# Autodesk Inventor assembly: embasev2
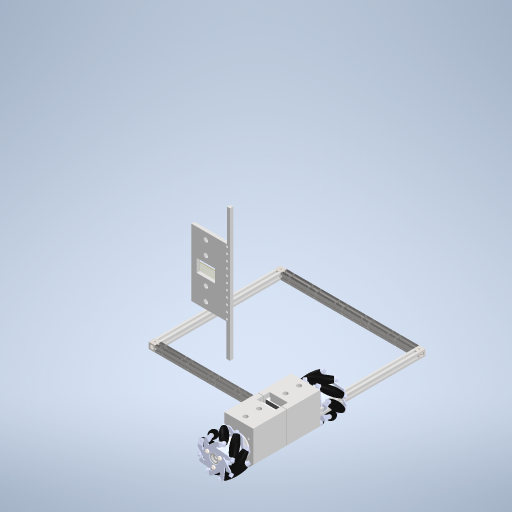
[picture p0: Inventor's stored thumbnail of the model, 512x512]
Saved by Autodesk Inventor 2024.2 (Build 282272000, 272)
## iProperties
Created: 2023-12-11
Part Number: embasev2
Document SubType Name: Assembly
Designer: adrie
Author: adrie
## Documents named in this file (24)
- C:\Users\eleves\Desktop\meca_robotbebou\embasev2\embasev2.iam
- C:\Users\eleves\Desktop\meca_robotbebou\embasev2\support_moteur_v3.ipt
- C:\Users\eleves\Desktop\meca_robotbebou\SF2423-10B41_MIR1.ipt
- C:\Users\eleves\Desktop\meca_robotbebou\60mm Double Aluminum Mecanum Wheel_MIR1.ipt
- C:\Users\eleves\Desktop\meca_robotbebou\moyeu_MIR1.ipt
- C:\Users\eleves\Desktop\meca_robotbebou\moyeu_end_MIR1.ipt
- C:\Users\eleves\Desktop\meca_robotbebou\embasev2\support_moteur_v3_MIR.ipt
- C:\Users\eleves\Desktop\meca_robotbebou\SF2423-10B41_MIR1_MIR.ipt
- C:\Users\eleves\Desktop\meca_robotbebou\60mm Double Aluminum Mecanum Wheel_MIR1_MIR.ipt
- C:\Users\eleves\Desktop\meca_robotbebou\moyeu_MIR1_MIR.ipt
- C:\Users\eleves\Desktop\meca_robotbebou\moyeu_end_MIR1_MIR.ipt
- C:\Users\eleves\Desktop\meca_robotbebou\SF2423-10B41_MIR1_MIR3.ipt
- C:\Users\eleves\Desktop\meca_robotbebou\60mm Double Aluminum Mecanum Wheel_MIR1_MIR3.ipt
- C:\Users\eleves\Desktop\meca_robotbebou\moyeu_MIR1_MIR3.ipt
- C:\Users\eleves\Desktop\meca_robotbebou\moyeu_end_MIR1_MIR3.ipt
- C:\Users\eleves\Desktop\meca_robotbebou\profile\MakerBeam-cube.ipt
- C:\Users\eleves\Desktop\meca_robotbebou\profile\profile210.ipt
- C:\Users\eleves\Desktop\meca_robotbebou\profile\profile190.ipt
- C:\Users\eleves\Desktop\meca_robotbebou\profile\MakerBeam-cube_MIR.ipt
- C:\Users\eleves\Desktop\meca_robotbebou\profile\MakerBeam-cube_MIR1.ipt
- C:\Users\eleves\Desktop\meca_robotbebou\profile\profile190_MIR.ipt
- C:\Users\eleves\Desktop\meca_robotbebou\profile\MakerBeam-cube_MIR_MIR.ipt
- C:\Users\eleves\Desktop\meca_robotbebou\profile\profile210_MIR.ipt
- C:\Users\eleves\Desktop\meca_robotbebou\embasev2\Pièce9.ipt
## Components (23 placed, 23 different names)
1. support_moteur_v3:1 — Placage:1, Placage:2, Angle:1
2. SF2423-10B41_MIR1:1 — Placage:1, Placage:2, Angle:1, Affleurement:1
3. 60mm Double Aluminum Mecanum Wheel_MIR1:1
4. moyeu_MIR1:1
5. moyeu_end_MIR1:1
6. support_moteur_v3_MIR:1 — Placage:3, Placage:4, Angle:2
7. SF2423-10B41_MIR1_MIR:1
8. 60mm Double Aluminum Mecanum Wheel_MIR1_MIR:1
9. moyeu_MIR1_MIR:1
10. moyeu_end_MIR1_MIR:1
11. SF2423-10B41_MIR1_MIR3:1 — Placage:3, Placage:4, Angle:2
12. 60mm Double Aluminum Mecanum Wheel_MIR1_MIR3:1
13. moyeu_MIR1_MIR3:1
14. moyeu_end_MIR1_MIR3:1
15. MakerBeam-cube:1
16. profile210:1
17. profile190:1
18. MakerBeam-cube_MIR:1
19. MakerBeam-cube_MIR1:1
20. profile190_MIR:1
21. MakerBeam-cube_MIR_MIR:1
22. profile210_MIR:1
23. Pièce9:1
## Relationships (19: Mate 7, Insert 6, Flush 4, Angle 2)
- [Insert]: 60mm Double Aluminum Mecanum Wheel_MIR1:1 ↔ moyeu_MIR1:1
- [Insert]: SF2423-10B41_MIR1:1 ↔ moyeu_MIR1:1
- [Insert]: 60mm Double Aluminum Mecanum Wheel_MIR1:1 ↔ moyeu_end_MIR1:1
- Placage:1 [Mate]: support_moteur_v3:1 ↔ SF2423-10B41_MIR1:1
- Placage:2 [Mate]: support_moteur_v3:1 ↔ SF2423-10B41_MIR1:1
- Angle:1 (0 deg): support_moteur_v3:1 ↔ SF2423-10B41_MIR1:1
- Affleurement:1 [Flush] (0.3 mm): SF2423-10B41_MIR1:1
- [Insert]: SF2423-10B41_MIR1_MIR3:1 ↔ moyeu_MIR1_MIR3:1
- [Insert]: 60mm Double Aluminum Mecanum Wheel_MIR1_MIR3:1 ↔ moyeu_MIR1_MIR3:1
- [Insert]: 60mm Double Aluminum Mecanum Wheel_MIR1_MIR3:1 ↔ moyeu_end_MIR1_MIR3:1
- Placage:3 [Mate]: support_moteur_v3_MIR:1 ↔ SF2423-10B41_MIR1_MIR3:1
- Placage:4 [Mate]: support_moteur_v3_MIR:1 ↔ SF2423-10B41_MIR1_MIR3:1
- Angle:2 (0 deg): support_moteur_v3_MIR:1 ↔ SF2423-10B41_MIR1_MIR3:1
- [Mate]: MakerBeam-cube:1 ↔ profile190:1
- [Flush]: MakerBeam-cube:1 ↔ profile190:1
- [Mate]: MakerBeam-cube:1 ↔ profile210:1
- [Flush]: MakerBeam-cube:1 ↔ profile210:1
- [Flush]: MakerBeam-cube_MIR1:1 ↔ profile190_MIR:1
- [Mate]: MakerBeam-cube_MIR1:1 ↔ profile190_MIR:1
